# Autodesk Inventor assembly: Red Alliance Bucket
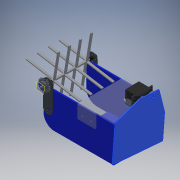
[picture p0: Inventor's stored thumbnail of the model, 180x180]
Saved by Autodesk Inventor 2016 (Build 200138000, 138)
## iProperties
Created: 2015-12-17
Part Number: Red Alliance Bucket
Document SubType Name: Assembly
Designer: TimB
Author: TimB
## Documents named in this file (14)
- C:\Users\TimB\Documents\GitHub\phi_robotics\3d-models\FTC_Tetrix_KOP_Block_Party\Tim Bloot Designs\JAr JaR Bot\Blue Alliance Bucket.iam
- C:\Users\TimB\Documents\GitHub\phi_robotics\3d-models\FTC_Tetrix_KOP_Block_Party\Tetrix_Kit_FTC\Autodesk Inventor Files\tetrix_739061_2012.ipt
- C:\Users\TimB\Documents\GitHub\phi_robotics\3d-models\FTC_Tetrix_KOP_Block_Party\Tim Bloot Designs\JAr JaR Bot\Bucket -  Top.ipt
- C:\Users\TimB\Documents\GitHub\phi_robotics\3d-models\FTC_Tetrix_KOP_Block_Party\Tetrix_Kit_FTC\Autodesk Inventor Files\tetrix_servo_mount.ipt
- C:\Users\TimB\Documents\GitHub\phi_robotics\3d-models\FTC_Tetrix_KOP_Block_Party\Tetrix_Kit_FTC\Autodesk Inventor Files\tetrix_servo_body.ipt
- C:\Users\TimB\Documents\GitHub\phi_robotics\3d-models\FTC_Tetrix_KOP_Block_Party\Tetrix_Kit_FTC\Autodesk Inventor Files\tetrix_bushing.ipt
- C:\Users\TimB\Documents\GitHub\phi_robotics\3d-models\FTC_Tetrix_KOP_Block_Party\Tim Bloot Designs\JAr JaR Bot\Bucket - Axle.ipt
- C:\Users\TimB\Documents\GitHub\phi_robotics\3d-models\FTC_Tetrix_KOP_Block_Party\Tim Bloot Designs\JAr JaR Bot\Bucket - 4 Rake.iam
- C:\Users\TimB\Documents\GitHub\phi_robotics\3d-models\FTC_Tetrix_KOP_Block_Party\Tetrix_Kit_FTC\Autodesk Inventor Files\tetrix_739092_2012.iam
- C:\Users\TimB\Documents\GitHub\phi_robotics\3d-models\FTC_Tetrix_KOP_Block_Party\Tetrix_Kit_FTC\Autodesk Inventor Files\tetrix_axle_lock.iam
- C:\Users\TimB\Documents\GitHub\phi_robotics\3d-models\FTC_Tetrix_KOP_Block_Party\Tetrix_Kit_FTC\Autodesk Inventor Files\tetrix_chain_gear-16t.ipt
- C:\Users\TimB\Documents\GitHub\phi_robotics\3d-models\FTC_Tetrix_KOP_Block_Party\Tim Bloot Designs\JAr JaR Bot\Bucket - BlueA.ipt
- C:\Users\TimB\Documents\GitHub\phi_robotics\3d-models\FTC_Tetrix_KOP_Block_Party\Tetrix_Kit_FTC\Autodesk Inventor Files\tetrix_servo_horn.iam
- C:\Users\TimB\Documents\GitHub\phi_robotics\3d-models\FTC_Tetrix_KOP_Block_Party\Tim Bloot Designs\JAr JaR Bot\Bucket - door 2.ipt
## Components (15 placed, 13 different names)
1. tetrix_739061_2012:1 — Rotational:2, Rigid:11
2. tetrix_739061_2012:2 — Rotational:1, Rigid:10
3. Bucket -  Top:1 — Rigid:4, Rigid:12
4. tetrix_bushing:1 — Rotational:2, Rotational:3
5. tetrix_bushing:2 — Rotational:1
6. tetrix_servo_mount:1 — Rigid:4, Rigid:5
7. tetrix_servo_body:1 — Rigid:5, Rotational:4
8. Bucket - Axle:1 — Rigid:6, Rigid:7, Rigid:9
9. Bucket - 4 Rake:1 [sub-assembly] — Rigid:7
10. tetrix_739092_2012:1 [sub-assembly] — Rigid:6, Rotational:3
11. tetrix_axle_lock:1 [sub-assembly] — Rigid:8, Rigid:9
12. tetrix_chain_gear-16t:1 — Rigid:8
13. Bucket - BlueA:1 — Rigid:10, Rigid:11, Rigid:12
14. tetrix_servo_horn:1 [sub-assembly] — Rigid:13, Rotational:4
15. Bucket - door 2:1 — Rigid:13
## Relationships (14: WeldJoint 10, RevoluteJoint 4)
- Rotational:1 [RevoluteJoint]: tetrix_739061_2012:2 ↔ tetrix_bushing:2
- Rotational:2 [RevoluteJoint]: tetrix_739061_2012:1 ↔ tetrix_bushing:1
- Rigid:4 [WeldJoint]: Bucket -  Top:1 ↔ tetrix_servo_mount:1
- Rigid:5 [WeldJoint]: tetrix_servo_mount:1 ↔ tetrix_servo_body:1
- Rigid:6 [WeldJoint]: Bucket - Axle:1 ↔ tetrix_739092_2012:1
- Rotational:3 [RevoluteJoint]: tetrix_bushing:1 ↔ tetrix_739092_2012:1
- Rigid:7 [WeldJoint] (-9.8 mm): Bucket - Axle:1 ↔ Bucket - 4 Rake:1
- Rigid:8 [WeldJoint]: tetrix_axle_lock:1 ↔ tetrix_chain_gear-16t:1
- Rigid:9 [WeldJoint] (-19.6 mm): Bucket - Axle:1 ↔ tetrix_axle_lock:1
- Rigid:10 [WeldJoint]: tetrix_739061_2012:2 ↔ Bucket - BlueA:1
- Rigid:11 [WeldJoint]: tetrix_739061_2012:1 ↔ Bucket - BlueA:1
- Rigid:12 [WeldJoint]: Bucket -  Top:1 ↔ Bucket - BlueA:1
- Rigid:13 [WeldJoint]: tetrix_servo_horn:1 ↔ Bucket - door 2:1
- Rotational:4 [RevoluteJoint]: tetrix_servo_body:1 ↔ tetrix_servo_horn:1
